# Autodesk Inventor assembly: assemblage
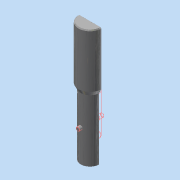
[picture p0: Inventor's stored thumbnail of the model, 180x180]
Saved by Autodesk Inventor 2017 (Build 210142000, 142)
## iProperties
Created: 2018-04-15
Part Number: assemblage
Document SubType Name: Assembly
Designer: RozierB
Author: RozierB
## Documents named in this file (4)
- D:\theo\système_ace\canon\20_ste_rma_1\assemblage.iam
- D:\theo\système_ace\canon\20_ste_rma_1\reservoir.ipt
- D:\theo\système_ace\canon\20_ste_rma_1\canon.ipt
- D:\theo\système_ace\canon\20_ste_rma_1\douille.ipt
## Components (3 placed, 3 different names)
1. reservoir:1 — Placage:5
2. canon:1 — Placage:2, Placage:3, Placage:4, Placage:5
3. douille:1 — Placage:2, Placage:3
## Relationships (4: Mate 4)
- Placage:2 [Mate]: canon:1 ↔ douille:1
- Placage:3 [Mate]: canon:1 ↔ douille:1
- Placage:4 [Mate]: canon:1
- Placage:5 [Mate]: reservoir:1 ↔ canon:1
